# Autodesk Inventor assembly: MECHENG334 2016 Bracket with pins
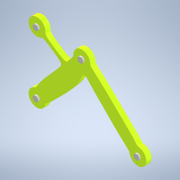
[picture p0: Inventor's stored thumbnail of the model, 180x180]
Saved by Autodesk Inventor 2021 (Build 250183000, 183)
## iProperties
Created: 2018-02-15
Part Number: MECHENG334 2016 Bracket with pins
Description: CAx-IF Rec.Pracs.---Model Styling and Organization---1.2---2011-12-15
Document SubType Name: Assembly
Designer: Jawal
Title: bracket.step
Sending System: 3D_Kernel_IO2017 Sp3 by CT CoreTechnologie
Preprocessor: STEP Interface 2017 Sp3 by CT CoreTechnologie
## Documents named in this file (3)
- C:\Users\Jawal\Documents\UNI\PART III\Semester 1\MECHENG 334\Project B\Calibration Data\MECHENG334 2016 Bracket with pins.iam
- C:\Users\Jawal\Documents\UNI\PART III\Semester 1\MECHENG 334\Project B\Calibration Data\BRACKET(2).ipt
- C:\Users\Jawal\Documents\UNI\PART III\Semester 1\MECHENG 334\Project B\Concept Design\pins.ipt
## Components (5 placed, 2 different names)
1. BRACKET(2)_1 — Rigid:1, Rigid:2, Rigid:3, Rigid:4
2. pins:2 — Rigid:3
3. pins:3 — Rigid:2
4. pins:4 — Rigid:4
5. pins:1 — Rigid:1
## Relationships (4: WeldJoint 4)
- Rigid:1 [WeldJoint]: BRACKET(2)_1 ↔ pins:1
- Rigid:2 [WeldJoint]: BRACKET(2)_1 ↔ pins:3
- Rigid:3 [WeldJoint]: BRACKET(2)_1 ↔ pins:2
- Rigid:4 [WeldJoint]: BRACKET(2)_1 ↔ pins:4
